# Autodesk Inventor assembly: Assembly1
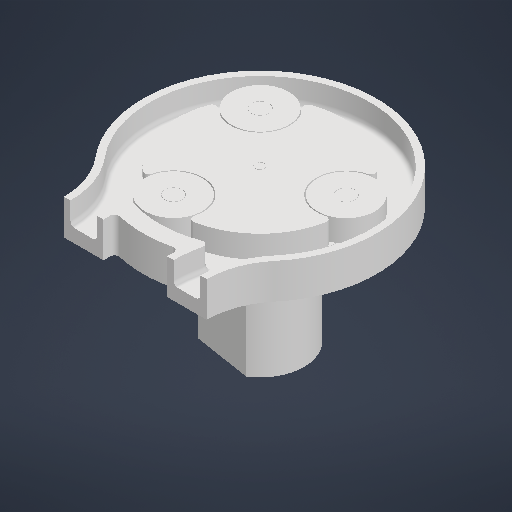
[picture p0: Inventor's stored thumbnail of the model, 512x512]
Saved by Autodesk Inventor 2026.2 (Build 302298000, 298)
## iProperties
Created: 2026-03-18
Part Number: Assembly1
Document SubType Name: Assembly
Designer: Cobble
Author: Cobble
## Documents named in this file (5)
- D:\Archive\Kreative Projekte\Obsidian\Online\Projects\Shot-Dispenser\Design V3\Assembly1.iam
- D:\Archive\Kreative Projekte\Obsidian\Online\Projects\Shot-Dispenser\Design V3\gewindeding.ipt
- D:\Archive\Kreative Projekte\Obsidian\Online\Projects\Shot-Dispenser\Design V3\Gehäuse.ipt
- D:\Archive\Kreative Projekte\Obsidian\Online\Projects\Shot-Dispenser\Design V3\Kugellager.ipt
- D:\Archive\Kreative Projekte\Obsidian\Online\Projects\Shot-Dispenser\Design V3\Pumpe.ipt
## Components (6 placed, 4 different names)
1. gewindeding:1 — Insert:1, Insert:2, Insert:3, Mate:1, Mate:2, Insert:4
2. Gehäuse:1 — Mate:1, Mate:2, Mate:3
3. Kugellager:1 — Insert:2
4. Kugellager:2 — Insert:3
5. Kugellager:3 — Insert:1
6. Pumpe:1 — Mate:3, Insert:4
## Relationships (7: Insert 4, Mate 3)
- Insert:1: gewindeding:1 ↔ Kugellager:3
- Insert:2: gewindeding:1 ↔ Kugellager:1
- Insert:3: gewindeding:1 ↔ Kugellager:2
- Mate:1: gewindeding:1 ↔ Gehäuse:1
- Mate:2: gewindeding:1 ↔ Gehäuse:1
- Mate:3: Gehäuse:1 ↔ Pumpe:1
- Insert:4: gewindeding:1 ↔ Pumpe:1
